# Autodesk Inventor assembly: POM_T5_08
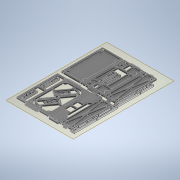
[picture p0: Inventor's stored thumbnail of the model, 180x180]
Saved by Autodesk Inventor 2022 (Build 260153000, 153)
## iProperties
Created: 2022-09-28
Part Number: POM_T5_08
Document SubType Name: Assembly
Designer: Masato
Author: Masato
## Documents named in this file (14)
- C:\Users\ヨコオリク\Documents\CITBrains\SUSTAINA-OP\Cam\POM_T5\POM_T5_08.iam
- C:\Users\ヨコオリク\Documents\CITBrains\SUSTAINA-OP\Cam\DisposableBoard.ipt
- C:\Users\ヨコオリク\Documents\CITBrains\SUSTAINA-OP\UpperBody\Cockpit\Cockpit_back_frame.ipt
- C:\Users\ヨコオリク\Documents\CITBrains\SUSTAINA-OP\UpperBody\Cockpit\Cockpit_battery_frame.ipt
- C:\Users\ヨコオリク\Documents\CITBrains\SUSTAINA-OP\UpperBody\Cockpit\Cockpit_carrier_board_frame.ipt
- C:\Users\ヨコオリク\Documents\CITBrains\SUSTAINA-OP\UpperBody\Cockpit\Cockpit_circuit_board_frame.ipt
- C:\Users\ヨコオリク\Documents\CITBrains\SUSTAINA-OP\UpperBody\Cockpit\Cockpit_front_frame.ipt
- C:\Users\ヨコオリク\Documents\CITBrains\SUSTAINA-OP\UpperBody\Cockpit\Cockpit_top_frame.ipt
- C:\Users\ヨコオリク\Documents\CITBrains\SUSTAINA-OP\OptionParts\DrillingJigs\Cockpit_back_frame_Jig.ipt
- C:\Users\ヨコオリク\Documents\CITBrains\SUSTAINA-OP\OptionParts\DrillingJigs\Cockpit_battery_back_door_Jig.ipt
- C:\Users\ヨコオリク\Documents\CITBrains\SUSTAINA-OP\OptionParts\DrillingJigs\Cockpit_battery_frame_Jig.ipt
- C:\Users\ヨコオリク\Documents\CITBrains\SUSTAINA-OP\OptionParts\DrillingJigs\Cockpit_carrier_board_frame_Jig.ipt
- C:\Users\ヨコオリク\Documents\CITBrains\SUSTAINA-OP\OptionParts\DrillingJigs\Cockpit_front_frame_Jig.ipt
- C:\Users\ヨコオリク\Documents\CITBrains\SUSTAINA-OP\OptionParts\DrillingJigs\Cockpit_side_frame_Jig.ipt
## Components (19 placed, 13 different names)
1. DisposableBoard:1 — フラッシュ:1, フラッシュ:2, フラッシュ:3, フラッシュ:4, フラッシュ:5, フラッシュ:8, フラッシュ:12
2. Cockpit_back_frame:1 — メイト:5, メイト:14, フラッシュ:10, フラッシュ:11, メイト:15, メイト:16, メイト:43, メイト:44
3. Cockpit_battery_frame:1 — メイト:4, フラッシュ:7, メイト:13, メイト:33, メイト:35
4. Cockpit_carrier_board_frame:1 — メイト:17, 正接:3, メイト:19, メイト:20, メイト:40, メイト:41
5. Cockpit_circuit_board_frame:1 — メイト:2, フラッシュ:5, フラッシュ:6, フラッシュ:8, メイト:12, フラッシュ:9, メイト:14, 正接:2, メイト:18, 正接:3, メイト:19, 正接:4, メイト:22, メイト:23, メイト:28, メイト:29
6. Cockpit_front_frame:1 — メイト:1, フラッシュ:9, フラッシュ:10, メイト:15
7. Cockpit_top_frame:1 — メイト:8, フラッシュ:6, フラッシュ:7, メイト:12, メイト:13
8. Cockpit_carrier_board_frame:2 — メイト:10, 正接:2, メイト:18, メイト:20, 正接:4, メイト:25, メイト:26
9. Cockpit_battery_frame:2 — メイト:6, フラッシュ:11, メイト:16, メイト:38, メイト:47
10. Cockpit_back_frame_Jig:1 — メイト:32, フラッシュ:12, メイト:33, メイト:34
11. Cockpit_battery_back_door_Jig:1 — メイト:27, メイト:28, メイト:29
12. Cockpit_battery_frame_Jig:1 — メイト:21, メイト:22, メイト:23
13. Cockpit_carrier_board_frame_Jig:1 — メイト:30, メイト:34, メイト:35, メイト:37
14. Cockpit_front_frame_Jig:1 — メイト:36, メイト:37, メイト:38, メイト:46
15. Cockpit_side_frame_Jig:1 — メイト:24, メイト:25, メイト:26
16. Cockpit_side_frame_Jig:2 — メイト:39, メイト:40, メイト:41
17. Cockpit_battery_frame_Jig:2 — メイト:45, メイト:46, メイト:47
18. Cockpit_battery_back_door_Jig:2 — メイト:42, メイト:43, メイト:44
19. Cockpit_battery_back_door_Jig:3
## Component patterns: (2 elements, first: Cockpit_battery_back_door_Jig:2)
## Relationships (57: Mate 42, Flush 12, Tangent 3)
- フラッシュ:1 [Flush]: DisposableBoard:1
- フラッシュ:2 [Flush]: DisposableBoard:1
- フラッシュ:3 [Flush]: DisposableBoard:1
- フラッシュ:4 [Flush]: DisposableBoard:1
- メイト:1 [Mate]: Cockpit_front_frame:1
- メイト:2 [Mate]: Cockpit_circuit_board_frame:1
- メイト:4 [Mate]: Cockpit_battery_frame:1
- メイト:5 [Mate]: Cockpit_back_frame:1
- メイト:6 [Mate]: Cockpit_battery_frame:2
- メイト:8 [Mate]: Cockpit_top_frame:1
- メイト:10 [Mate]: Cockpit_carrier_board_frame:2
- フラッシュ:5 [Flush] (-2 mm): DisposableBoard:1 ↔ Cockpit_circuit_board_frame:1
- フラッシュ:6 [Flush]: Cockpit_circuit_board_frame:1 ↔ Cockpit_top_frame:1
- フラッシュ:7 [Flush]: Cockpit_battery_frame:1 ↔ Cockpit_top_frame:1
- フラッシュ:8 [Flush] (-2 mm): DisposableBoard:1 ↔ Cockpit_circuit_board_frame:1
- メイト:12 [Mate] (2.1 mm): Cockpit_circuit_board_frame:1 ↔ Cockpit_top_frame:1
- メイト:13 [Mate] (2.1 mm): Cockpit_battery_frame:1 ↔ Cockpit_top_frame:1
- フラッシュ:9 [Flush]: Cockpit_circuit_board_frame:1 ↔ Cockpit_front_frame:1
- メイト:14 [Mate] (2.1 mm): Cockpit_back_frame:1 ↔ Cockpit_circuit_board_frame:1
- フラッシュ:10 [Flush]: Cockpit_back_frame:1 ↔ Cockpit_front_frame:1
- フラッシュ:11 [Flush]: Cockpit_back_frame:1 ↔ Cockpit_battery_frame:2
- メイト:15 [Mate] (2.1 mm): Cockpit_back_frame:1 ↔ Cockpit_front_frame:1
- メイト:16 [Mate] (2.1 mm): Cockpit_back_frame:1 ↔ Cockpit_battery_frame:2
- メイト:17 [Mate]: Cockpit_carrier_board_frame:1
- 正接:2 [Tangent] (2.1 mm): Cockpit_circuit_board_frame:1 ↔ Cockpit_carrier_board_frame:2
- メイト:18 [Mate] (2.1 mm): Cockpit_circuit_board_frame:1 ↔ Cockpit_carrier_board_frame:2
- 正接:3 [Tangent] (2.1 mm): Cockpit_carrier_board_frame:1 ↔ Cockpit_circuit_board_frame:1
- メイト:19 [Mate] (2.1 mm): Cockpit_carrier_board_frame:1 ↔ Cockpit_circuit_board_frame:1
- メイト:20 [Mate] (2.1 mm): Cockpit_carrier_board_frame:1 ↔ Cockpit_carrier_board_frame:2
- 正接:4 [Tangent] (2.1 mm): Cockpit_circuit_board_frame:1 ↔ Cockpit_carrier_board_frame:2
- メイト:21 [Mate]: Cockpit_battery_frame_Jig:1
- メイト:22 [Mate] (2.1 mm): Cockpit_circuit_board_frame:1 ↔ Cockpit_battery_frame_Jig:1
- メイト:23 [Mate] (2.1 mm): Cockpit_circuit_board_frame:1 ↔ Cockpit_battery_frame_Jig:1
- メイト:24 [Mate]: Cockpit_side_frame_Jig:1
- メイト:25 [Mate] (2.1 mm): Cockpit_carrier_board_frame:2 ↔ Cockpit_side_frame_Jig:1
- メイト:26 [Mate] (2.1 mm): Cockpit_carrier_board_frame:2 ↔ Cockpit_side_frame_Jig:1
- メイト:27 [Mate]: Cockpit_battery_back_door_Jig:1
- メイト:28 [Mate] (2.1 mm): Cockpit_circuit_board_frame:1 ↔ Cockpit_battery_back_door_Jig:1
- メイト:29 [Mate] (2.1 mm): Cockpit_circuit_board_frame:1 ↔ Cockpit_battery_back_door_Jig:1
- メイト:30 [Mate]: Cockpit_carrier_board_frame_Jig:1
- メイト:32 [Mate]: Cockpit_back_frame_Jig:1
- フラッシュ:12 [Flush] (2 mm): DisposableBoard:1 ↔ Cockpit_back_frame_Jig:1
- メイト:33 [Mate] (2.1 mm): Cockpit_battery_frame:1 ↔ Cockpit_back_frame_Jig:1
- メイト:34 [Mate] (2.1 mm): Cockpit_back_frame_Jig:1 ↔ Cockpit_carrier_board_frame_Jig:1
- メイト:35 [Mate] (2.1 mm): Cockpit_battery_frame:1 ↔ Cockpit_carrier_board_frame_Jig:1
- メイト:36 [Mate]: Cockpit_front_frame_Jig:1
- メイト:37 [Mate] (2.1 mm): Cockpit_carrier_board_frame_Jig:1 ↔ Cockpit_front_frame_Jig:1
- メイト:38 [Mate] (2.1 mm): Cockpit_battery_frame:2 ↔ Cockpit_front_frame_Jig:1
- メイト:39 [Mate]: Cockpit_side_frame_Jig:2
- メイト:40 [Mate] (2.1 mm): Cockpit_carrier_board_frame:1 ↔ Cockpit_side_frame_Jig:2
- メイト:41 [Mate] (2.1 mm): Cockpit_carrier_board_frame:1 ↔ Cockpit_side_frame_Jig:2
- メイト:42 [Mate]: Cockpit_battery_back_door_Jig:2
- メイト:43 [Mate] (2.1 mm): Cockpit_back_frame:1 ↔ Cockpit_battery_back_door_Jig:2
- メイト:44 [Mate] (2.1 mm): Cockpit_back_frame:1 ↔ Cockpit_battery_back_door_Jig:2
- メイト:45 [Mate]: Cockpit_battery_frame_Jig:2
- メイト:46 [Mate] (2.1 mm): Cockpit_front_frame_Jig:1 ↔ Cockpit_battery_frame_Jig:2
- メイト:47 [Mate] (2.1 mm): Cockpit_battery_frame:2 ↔ Cockpit_battery_frame_Jig:2
